# Autodesk Inventor assembly: chest
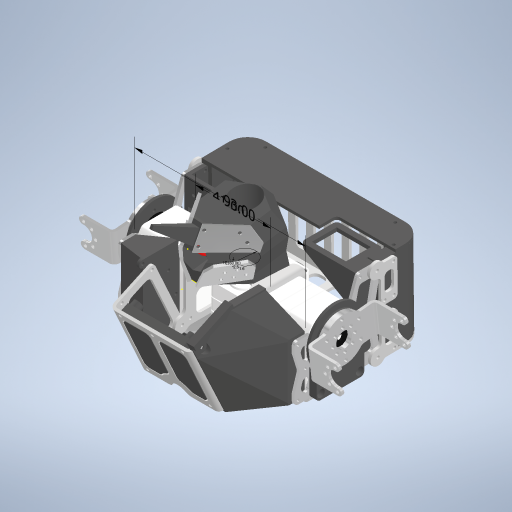
[picture p0: Inventor's stored thumbnail of the model, 512x512]
Saved by Autodesk Inventor 2024.1 (Build 281209000, 209)
## iProperties
Created: 2024-02-14
Part Number: chest
Document SubType Name: Assembly
Designer: hibik
Author: hibik
## Documents named in this file (13)
- C:\Users\hibik\Documents\Robomech\HR\Eglantyne\hard\upper_body\chest.iam
- C:\Users\hibik\Documents\Robomech\HR\Eglantyne\hard\under_body\waist.iam
- C:\Users\hibik\Documents\Robomech\HR\Eglantyne\hard\upper_body\sholder.iam
- C:\Users\hibik\Documents\Robomech\HR\Eglantyne\hard\upper_body\sholder_joint_cover.ipt
- C:\Users\hibik\Documents\Robomech\HR\Eglantyne\hard\upper_body\neck_bace.ipt
- C:\Users\hibik\Documents\Robomech\HR\Eglantyne\hard\upper_body\board_cover_top.ipt
- C:\Users\hibik\Documents\Robomech\HR\Eglantyne\hard\upper_body\board_cover_inside.ipt
- C:\Users\hibik\Documents\Robomech\HR\Eglantyne\hard\upper_body\board_cover_side.ipt
- C:\Users\hibik\Documents\Robomech\HR\Eglantyne\hard\upper_body\board_cover_side_right.ipt
- C:\Users\hibik\Documents\Robomech\HR\Eglantyne\hard\head\head.iam
- C:\Users\hibik\Documents\Robomech\HR\Eglantyne\hard\upper_body\chest_cover.iam
- C:\Users\hibik\Documents\Robomech\HR\Eglantyne\hard\upper_body\bluetooth_setter.ipt
- C:\Users\hibik\Documents\Robomech\HR\Eglantyne\hard\upper_body\button_setter.ipt
## Components (14 placed, 12 different names)
1. waist:1 [sub-assembly] — 挿入:1, 挿入:2, 挿入:3, 挿入:4, 挿入:5, 挿入:6, メイト:2, 挿入:8, 角度:1, メイト:5, メイト:6, メイト:7, 挿入:12, 挿入:13, 挿入:16, 挿入:17, フラッシュ:4, 挿入:18, フラッシュ:5
2. sholder:1 [sub-assembly] — 挿入:2
3. sholder_joint_cover:1 — 挿入:3, 挿入:4
4. sholder:2 [sub-assembly] — 挿入:1
5. sholder_joint_cover:2 — 挿入:5, 挿入:6
6. neck_bace:1 — メイト:2, 挿入:8, 角度:1, 挿入:9, 挿入:14
7. board_cover_top:1 — 挿入:9, メイト:3, フラッシュ:3, メイト:4
8. board_cover_inside:1 — メイト:3, フラッシュ:3, メイト:4
9. board_cover_side:1 — メイト:5, メイト:6, メイト:7
10. board_cover_side_right:1 — 挿入:12, 挿入:13
11. head:1 [sub-assembly] — 挿入:14
12. chest_cover:1 [sub-assembly] — 挿入:16
13. bluetooth_setter:1 — 挿入:17, フラッシュ:4
14. button_setter:1 — 挿入:18, フラッシュ:5
## Relationships (24: Insert 14, Mate 6, Flush 3, Angle 1)
- 挿入:1 [Insert]: waist:1 ↔ sholder:2
- 挿入:2 [Insert]: waist:1 ↔ sholder:1
- 挿入:3 [Insert]: waist:1 ↔ sholder_joint_cover:1
- 挿入:4 [Insert]: waist:1 ↔ sholder_joint_cover:1
- 挿入:5 [Insert]: waist:1 ↔ sholder_joint_cover:2
- 挿入:6 [Insert]: waist:1 ↔ sholder_joint_cover:2
- メイト:2 [Mate]: waist:1 ↔ neck_bace:1
- 挿入:8 [Insert]: waist:1 ↔ neck_bace:1
- 角度:1 [Angle] (0 deg): waist:1 ↔ neck_bace:1
- 挿入:9 [Insert]: neck_bace:1 ↔ board_cover_top:1
- メイト:3 [Mate]: board_cover_top:1 ↔ board_cover_inside:1
- フラッシュ:3 [Flush]: board_cover_top:1 ↔ board_cover_inside:1
- メイト:4 [Mate] (2 mm): board_cover_top:1 ↔ board_cover_inside:1
- メイト:5 [Mate]: waist:1 ↔ board_cover_side:1
- メイト:6 [Mate]: waist:1 ↔ board_cover_side:1
- メイト:7 [Mate]: waist:1 ↔ board_cover_side:1
- 挿入:12 [Insert]: waist:1 ↔ board_cover_side_right:1
- 挿入:13 [Insert]: waist:1 ↔ board_cover_side_right:1
- 挿入:14 [Insert]: neck_bace:1 ↔ head:1
- 挿入:16 [Insert]: waist:1 ↔ chest_cover:1
- 挿入:17 [Insert]: waist:1 ↔ bluetooth_setter:1
- フラッシュ:4 [Flush]: waist:1 ↔ bluetooth_setter:1
- 挿入:18 [Insert]: waist:1 ↔ button_setter:1
- フラッシュ:5 [Flush]: waist:1 ↔ button_setter:1
